# Autodesk Inventor assembly: midlleslide
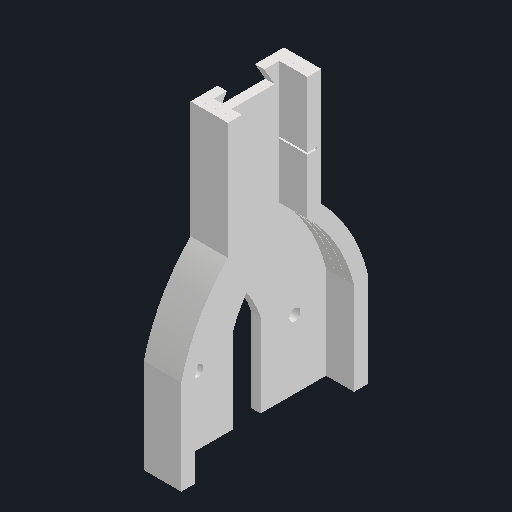
[picture p0: Inventor's stored thumbnail of the model, 512x512]
Saved by Autodesk Inventor 2026.2 (Build 302298000, 298)
## iProperties
Created: 2026-04-17
Part Number: midlleslide
Document SubType Name: Assembly
Designer: danda
Author: danda
## Documents named in this file (4)
- C:\Users\danda\BOM-project\Project\CAD\sorting\middleslide\midlleslide.iam
- C:\Users\danda\BOM-project\Project\CAD\sorting\middleslide\middlelsidewall.ipt
- C:\Users\danda\BOM-project\Project\CAD\sorting\middleslide\middleslidestick.ipt
- C:\Users\danda\BOM-project\Project\CAD\sorting\middleslide\newmiddle.ipt
## Components (8 placed, 3 different names)
1. middleslidestick:1 — Mate:29, Flush:15, Mate:35
2. middleslidestick:2 — Mate:22, Mate:23, Mate:24, Mate:25, Mate:26, Mate:27, Mate:28, Flush:16, Mate:34
3. middleslidestick:3 — Mate:31, Mate:32, Flush:14
4. middleslidestick:4 — Mate:30, Flush:17, Mate:33
5. middlelsidewall:1 — Mate:21, Flush:10, Flush:11, Flush:12, Flush:13, Mate:22, Mate:25, Mate:36
6. middlelsidewall:2 — Mate:20, Mate:21, Flush:10, Flush:12, Mate:23, Mate:26
7. middlelsidewall:3 — Mate:20, Flush:11, Flush:13, Mate:24, Mate:27
8. newmiddle:1 — Mate:28, Mate:29, Mate:30, Mate:31, Mate:32, Flush:14, Flush:15, Flush:16, Flush:17, Mate:33, Mate:34, Mate:35, Mate:36
## Relationships (25: Mate 17, Flush 8)
- Mate:20: middlelsidewall:2 ↔ middlelsidewall:3
- Mate:21: middlelsidewall:1 ↔ middlelsidewall:2
- Flush:10: middlelsidewall:1 ↔ middlelsidewall:2
- Flush:11: middlelsidewall:1 ↔ middlelsidewall:3
- Flush:12: middlelsidewall:1 ↔ middlelsidewall:2
- Flush:13: middlelsidewall:1 ↔ middlelsidewall:3
- Mate:22: middleslidestick:2 ↔ middlelsidewall:1
- Mate:23: middleslidestick:2 ↔ middlelsidewall:2
- Mate:24: middleslidestick:2 ↔ middlelsidewall:3
- Mate:25: middleslidestick:2 ↔ middlelsidewall:1
- Mate:26: middleslidestick:2 ↔ middlelsidewall:2
- Mate:27: middleslidestick:2 ↔ middlelsidewall:3
- Mate:28: middleslidestick:2 ↔ newmiddle:1
- Mate:29: middleslidestick:1 ↔ newmiddle:1
- Mate:30: middleslidestick:4 ↔ newmiddle:1
- Mate:31: middleslidestick:3 ↔ newmiddle:1
- Mate:32: middleslidestick:3 ↔ newmiddle:1
- Flush:14: middleslidestick:3 ↔ newmiddle:1
- Flush:15: middleslidestick:1 ↔ newmiddle:1
- Flush:16: middleslidestick:2 ↔ newmiddle:1
- Flush:17: middleslidestick:4 ↔ newmiddle:1
- Mate:33: middleslidestick:4 ↔ newmiddle:1
- Mate:34: middleslidestick:2 ↔ newmiddle:1
- Mate:35: middleslidestick:1 ↔ newmiddle:1
- Mate:36: middlelsidewall:1 ↔ newmiddle:1
